# Autodesk Inventor assembly: CRBT155A
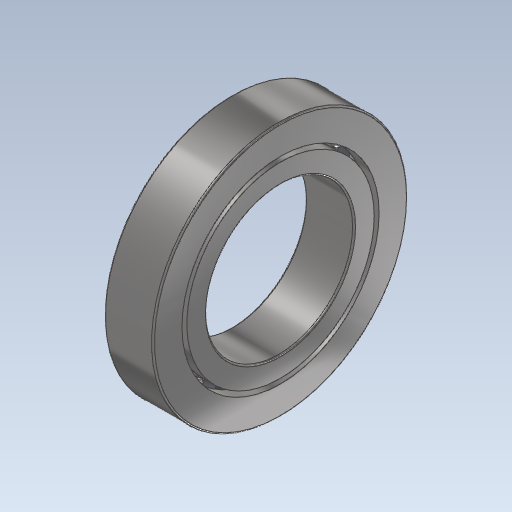
[picture p0: Inventor's stored thumbnail of the model, 512x512]
Saved by Autodesk Inventor 2024 (Build 280153000, 153)
## iProperties
Category: PARTsolutions
Company: IKO
Created: 2023-09-04
Part Number: CRBT155A
Catalog Web Link: www.cadenas.de
Description: Ultra Slim Type Crossed Roller Bearings (CRBT...A)-
Vendor: IKO
Document SubType Name: Assembly
Designer: psAdmin
Manufacturer: IKO
Mass: 1.59961 g
Surface Area: 24.8189 cm^2
Volume: 1.59961 cm^3
Density: 1 g/cm^3
PSOL_IDENT_0: {$CADENAS_DATA/23d-libs/iko/iko_bearings/crossed_rb/ultra_slim_type_crb/ultra_slim_type_crbt.prj},20
PSOL_IDENT_1: 1 {VTYP=3D},{NB=CRBT155A},{LINA=CRBT155A},{NN=Ultra Slim Type Crossed Roller Bearings (CRBT...A)},{D
PSOL_IDENT_2: ATE=09.07.2020 23:28:49},{GEOMDATE=08.07.2020 06:24:28},{VERSION=},{LINEID=220},{WBVAR=},{WBNUMERIC=
PSOL_IDENT_3: }  {NB=CRBT155A},{LINA=CRBT155A},{KT=DUMMY},{IDNR=},{STDRT=15},{ORDER=CRBT155A},{MASS=11.9},{SD=15},
PSOL_IDENT_4: {D=26},{B=5},{SR=0.15},{SDA=17.5},{DA=22.0},{DAR=2.0},{ZEFF=16},{RS=0.3},{DETC=1.6},{PCDRL=19.6},{SD
PSOL_IDENT_5: OR=20.10},{DIRR=19.10},{COG=0.0},{SDOG=0.0},{OH=0.0},{NH=0},{CR=1320},{COR=1110},{SC=0},{N=8},{N1=1.
PSOL_IDENT_6: 67}
NB: CRBT155A
NN: Ultra Slim Type Crossed Roller Bearings (CRBT...A)
NBSYN: $ORDER.
LINA: CRBT155A
CATALOG: IKO (Nippon Thompson
STDRT: 15
ORDER: CRBT155A
MASS: 11.9
SD: 15
D: 26
B: 5
SR: 0.15
SDA: 17.5
DA: 22
CR: 1320
COR: 1110
SUPPLIER: IKO
ARTICLENO: CRBT155A
BOMINFO: CRBT155A
CREATOR: CADENAS GmbH
Title: CRBT155A
Author: Cadenas PARTsolutions
## Documents named in this file (7)
- C:\Users\michi\OneDrive - Kyoto University\lab\6_SHINOBI\FUHGA4\Design_Mechanism\5_birdeye\birdeye_shoulderUnit\_CRBT155A.iam
- C:\Users\michi\OneDrive - Kyoto University\lab\6_SHINOBI\FUHGA4\Design_Mechanism\5_birdeye\birdeye_shoulderUnit\IKO_CRBT155A\AIS2024\CRBT155A_PART1.ipt
- C:\Users\michi\OneDrive - Kyoto University\lab\6_SHINOBI\FUHGA4\Design_Mechanism\5_birdeye\birdeye_shoulderUnit\IKO_CRBT155A\AIS2024\CRBT155A_PART2.ipt
- C:\Users\michi\OneDrive - Kyoto University\lab\6_SHINOBI\FUHGA4\Design_Mechanism\5_birdeye\birdeye_shoulderUnit\IKO_CRBT155A\AIS2024\CRBT155A_PART3.ipt
- C:\Users\michi\OneDrive - Kyoto University\lab\6_SHINOBI\FUHGA4\Design_Mechanism\5_birdeye\birdeye_shoulderUnit\IKO_CRBT155A\AIS2024\CRBT155A_PART4.ipt
- C:\Users\michi\OneDrive - Kyoto University\lab\6_SHINOBI\FUHGA4\Design_Mechanism\5_birdeye\birdeye_shoulderUnit\IKO_CRBT155A\AIS2024\CRBT155A_PART5.ipt
- C:\Users\michi\OneDrive - Kyoto University\lab\6_SHINOBI\FUHGA4\Design_Mechanism\5_birdeye\birdeye_shoulderUnit\IKO_CRBT155A\AIS2024\CRBT155A_PART6.ipt
## Components (34 placed, 6 different names)
1. CRBT155A_PART1:1 — メイト:1, フラッシュ:1
2. CRBT155A_PART2:1 — メイト:1, フラッシュ:1
3. CRBT155A_PART3:1
4. CRBT155A_PART3:2
5. CRBT155A_PART3:3
6. CRBT155A_PART3:4
7. CRBT155A_PART3:5
8. CRBT155A_PART3:6
9. CRBT155A_PART3:7
10. CRBT155A_PART3:8
11. CRBT155A_PART4:1
12. CRBT155A_PART4:2
13. CRBT155A_PART4:3
14. CRBT155A_PART4:4
15. CRBT155A_PART4:5
16. CRBT155A_PART4:6
17. CRBT155A_PART4:7
18. CRBT155A_PART4:8
19. CRBT155A_PART5:1
20. CRBT155A_PART5:2
21. CRBT155A_PART5:3
22. CRBT155A_PART5:4
23. CRBT155A_PART5:5
24. CRBT155A_PART5:6
25. CRBT155A_PART5:7
26. CRBT155A_PART5:8
27. CRBT155A_PART6:1
28. CRBT155A_PART6:2
29. CRBT155A_PART6:3
30. CRBT155A_PART6:4
31. CRBT155A_PART6:5
32. CRBT155A_PART6:6
33. CRBT155A_PART6:7
34. CRBT155A_PART6:8
## Relationships (2: Mate 1, Flush 1)
- メイト:1 [Mate]: CRBT155A_PART1:1 ↔ CRBT155A_PART2:1
- フラッシュ:1 [Flush]: CRBT155A_PART1:1 ↔ CRBT155A_PART2:1
